# Autodesk Inventor assembly: Box Arm
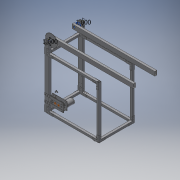
[picture p0: Inventor's stored thumbnail of the model, 180x180]
Saved by Autodesk Inventor 2018 (Build 220112000, 112)
## iProperties
Created: 2019-01-16
Part Number: Box Arm
Document SubType Name: Assembly
Designer: Gabriel
Author: Gabriel
## Documents named in this file (33)
- C:\Users\Gabriel\Documents\GitHub\2019CAD\Drivebase Box Arm\Box Arm.iam
- C:\Users\Gabriel\Documents\GitHub\2019CAD\Drivebase Box Arm\30in 1x1 Beam.ipt
- C:\Users\Gabriel\Documents\GitHub\2019CAD\Drivebase Box Arm\25in 1x1 Beam.ipt
- C:\Users\Gabriel\Documents\GitHub\2019CAD\Drivebase Box Arm\17in 1x1 Beam.ipt
- C:\Users\Gabriel\Documents\GitHub\2019CAD\Drivebase Box Arm\23in 1x1 Beam.ipt
- C:\Users\Gabriel\Documents\GitHub\2019CAD\Drivebase Box Arm\L gusset.ipt
- C:\Users\Gabriel\Documents\GitHub\2019CAD\Drivebase Box Arm\34.48in Arm Bea.ipt
- C:\Users\Gabriel\Documents\GitHub\2019CAD\Drivebase Box Arm\0_500_ID_x_1_125_OD_x_0_313_WD_Flanged_Bearing_217-2731.ipt
- C:\Users\Gabriel\Documents\GitHub\2019CAD\Drivebase Box Arm\_72t_Aluminum_Plate_Sprocket_25_Chain_1-1_8_Bearing_Bore_217-2627.ipt
- C:\Users\Gabriel\Documents\GitHub\2019CAD\Drivebase Box Arm\Hex Hub.ipt
- C:\Users\Gabriel\Documents\GitHub\2019CAD\Drivebase Box Arm\0.5in Hex Shaft.ipt
- C:\Users\Gabriel\Documents\GitHub\2019CAD\Drivebase Box Arm\1_2_Acetal_Spacer_-_1_2_Hex_217-3261.ipt
- C:\Users\Gabriel\Documents\GitHub\2019CAD\Drivebase Box Arm\am-0150 Toughbox Large Output Gear.ipt
- C:\Users\Gabriel\Documents\GitHub\2019CAD\Drivebase Box Arm\Mini_CIM_Motor_217-3371.ipt
- C:\Users\Gabriel\Documents\GitHub\2019CAD\Drivebase Box Arm\ARm Gearbox Plate.ipt
- C:\Users\Gabriel\Documents\GitHub\2019CAD\Drivebase Box Arm\1_16_Acetal_Spacer_-_1_2_Hex_217-3257.ipt
- C:\Users\Gabriel\Documents\GitHub\2019CAD\Drivebase Box Arm\3_8in Hex Shaft.ipt
- C:\Users\Gabriel\Documents\GitHub\2019CAD\Drivebase Box Arm\10T_Steel_Spur_Gear_20_DP_12T_Center_Distance_CIM_Motor_217-6334.ipt
- C:\Users\Gabriel\Documents\GitHub\2019CAD\Drivebase Box Arm\am-0143 50 Tooth 20 dp Aluminum Gear 375 Hex.ipt
- C:\Users\Gabriel\Documents\GitHub\2019CAD\Drivebase Box Arm\am-0151 14T 20dp 375hex.ipt
- C:\Users\Gabriel\Documents\GitHub\2019CAD\Drivebase Box Arm\1_16_Acetal_Spacer_-_3_8_Hex_217-3258.ipt
- C:\Users\Gabriel\Documents\GitHub\2019CAD\Drivebase Box Arm\40t_Aluminum_Spur_Gear_20_DP_3_8_Hex_Bore_217-2707.ipt
- C:\Users\Gabriel\Documents\GitHub\2019CAD\Drivebase Box Arm\am-0028 00.375'' id Flanged, Shielded Ball Bearing (FR6ZZ).ipt
- C:\Users\Gabriel\Documents\GitHub\2019CAD\Drivebase Box Arm\92196A271_18-8 STAINLESS STEEL SOCKET HEAD CAP SCREW.ipt
- C:\Users\Gabriel\Documents\GitHub\2019CAD\Drivebase Box Arm\am-3621 - S25-18HA-500H.ipt
- C:\Users\Gabriel\Documents\GitHub\2019CAD\Drivebase Box Arm\Clamping_Shaft_Collar_-_1_2_Hex_ID_217-2737.ipt
- C:\Users\Gabriel\Documents\GitHub\2019CAD\Drivebase Box Arm\#10 Washer.ipt
- C:\Users\Gabriel\Downloads\3D Model Spacer.ipt
- C:\Users\Gabriel\Downloads\Gearbox Mounting Gusset.ipt
- C:\Users\Gabriel\Downloads\92196A251_18-8 STAINLESS STEEL SOCKET HEAD CAP SCREW.ipt
- C:\Users\Gabriel\Downloads\91831A011_TYPE 18-8 STAINLESS STL NYLON-INSERT LOCKNUT.ipt
- C:\Users\Gabriel\Downloads\Churro For ARm Gearbox.ipt
- C:\Users\Gabriel\Downloads\92196A245_18-8 STAINLESS STEEL SOCKET HEAD CAP SCREW.ipt
## Components (119 placed, 32 different names)
1. 30in 1x1 Beam:1 — Mate:13, Mate:14, Mate:37, Mate:38, Mate:74, Mate:75, Mate:83, Mate:84, Mate:98, Mate:99, Mate:101, Mate:102, Mate:103, Mate:104
2. 30in 1x1 Beam:2 — Mate:11, Mate:12, Mate:39, Mate:40, Mate:73, Mate:76, Mate:86, Mate:87, Mate:95, Mate:96, Mate:105, Mate:106, Mate:107, Mate:108, Mate:441, Mate:442, Mate:457, Mate:458, Mate:459, Mate:460, Mate:461, Mate:462, Mate:497
3. 25in 1x1 Beam:1 — Mate:512, Mate:513, Mate:514, Mate:515, Mate:516, Mate:517, Mate:518, Mate:519, Mate:520, Mate:521
4. 25in 1x1 Beam:2 — Mate:464, Mate:465, Mate:466, Mate:467, Mate:469, Mate:472, Mate:475, Mate:476, Mate:477, Mate:478, Mate:479, Mate:480, Mate:481, Mate:482, Mate:487
5. 25in 1x1 Beam:3 — Mate:496, Mate:497, Mate:498, Mate:499, Mate:500, Mate:501, Mate:502, Mate:503, Mate:504
6. 25in 1x1 Beam:4 — Mate:31, Mate:32, Mate:55, Mate:56, Mate:100, Mate:505, Mate:512
7. 17in 1x1 Beam:1 — Mate:504, Mate:505, Mate:506, Mate:507, Mate:508, Mate:509, Mate:510, Mate:511
8. 17in 1x1 Beam:2 — Mate:21, Mate:22, Mate:23, Mate:24
9. 23in 1x1 Beam:1 — Mate:483, Mate:484, Mate:485, Mate:486, Mate:487, Mate:488, Mate:489, Mate:490, Mate:491, Mate:492, Mate:493, Mate:494, Mate:495
10. 23in 1x1 Beam:2 — Mate:47, Mate:48, Mate:51, Mate:52, Mate:85, Mate:89, Mate:522, Mate:523, Mate:524, Mate:525
11. L gusset:1 — Mate:466, Mate:469, Mate:476, Mate:498, Mate:500, Mate:501, Mate:570, Mate:571
12. L gusset:4 — Mate:465, Mate:477, Mate:478, Mate:479, Mate:483, Mate:488, Mate:489, Mate:526, Mate:527, Mate:566, Mate:567, Mate:568, Mate:569
13. L gusset:5 — Mate:51, Mate:52, Mate:513, Mate:517, Mate:518, Mate:519
14. L gusset:7 — Mate:11, Mate:12, Mate:23, Mate:24
15. L gusset:9 — Mate:13, Mate:14, Mate:21, Mate:22
16. L gusset:11 — Mate:31, Mate:32, Mate:74, Mate:75
17. L gusset:12 — Mate:73, Mate:76, Mate:499, Mate:502, Mate:503
18. L gusset:13 — Mate:485, Mate:490, Mate:491
19. L gusset:14 — Mate:47, Mate:48
20. L gusset:15 — Mate:39, Mate:40, Mate:77, Mate:80
21. L gusset:16 — Mate:37, Mate:38, Mate:78, Mate:79
22. L gusset:17 — Mate:55, Mate:56, Mate:515, Mate:520, Mate:521
23. L gusset:18 — Mate:467, Mate:472, Mate:475, Mate:496, Mate:507, Mate:508, Mate:509
24. L gusset:19 — Mate:506, Mate:510, Mate:511, Mate:516
25. 17in 1x1 Beam:3 — Mate:77, Mate:78, Mate:79, Mate:80
26. 34.48in Arm Bea:2 — Mate:109, Mate:110
27. 0_500_ID_x_1_125_OD_x_0_313_WD_Flanged_Bearing_217-2731:1 — Mate:103, Mate:104, Mate:139, Mate:140, Mate:149
28. 0_500_ID_x_1_125_OD_x_0_313_WD_Flanged_Bearing_217-2731:2 — Mate:107, Mate:108, Mate:126, Mate:152
29. 0_500_ID_x_1_125_OD_x_0_313_WD_Flanged_Bearing_217-2731:5 — Mate:101, Mate:102, Mate:143
30. 0_500_ID_x_1_125_OD_x_0_313_WD_Flanged_Bearing_217-2731:8 — Mate:105, Mate:106, Mate:446, Mate:447
31. L gusset:20 — Mate:464, Mate:480, Mate:481, Mate:482, Mate:484, Mate:494, Mate:495, Mate:557
32. L gusset:21 — Mate:89, Mate:514, Mate:522, Mate:523
33. L gusset:22 — Mate:98, Mate:99, Mate:100
34. L gusset:23 — Mate:95, Mate:96
35. L gusset:24 — Mate:83, Mate:84, Mate:85, Mate:524, Mate:525
36. L gusset:25 — Mate:86, Mate:87, Mate:486, Mate:492, Mate:493
37. _72t_Aluminum_Plate_Sprocket_25_Chain_1-1_8_Bearing_Bore_217-2627:2 — Mate:120, Mate:121, Mate:138, Flush:4
38. Hex Hub:2 — Mate:109, Mate:110, Mate:111, Mate:112, Mate:113
39. Hex Hub:3 — Mate:120, Mate:121, Mate:138, Mate:444, Mate:445
40. 1_2_Acetal_Spacer_-_1_2_Hex_217-3261:1 — Mate:126, Mate:406
41. 1_2_Acetal_Spacer_-_1_2_Hex_217-3261:3 — Mate:111, Mate:112, Mate:113
42. 34.48in Arm Bea:3 — Mate:128
43. Hex Hub:4 — Mate:136, Mate:139, Mate:140
44. Hex Hub:5 — Mate:128, Mate:133
45. 1_2_Acetal_Spacer_-_1_2_Hex_217-3261:7 — Mate:143, Mate:403
46. 1_2_Acetal_Spacer_-_1_2_Hex_217-3261:8 — Mate:133, Mate:136
47. 1_2_Acetal_Spacer_-_1_2_Hex_217-3261:9 — Mate:149
48. 1_2_Acetal_Spacer_-_1_2_Hex_217-3261:10 — Mate:152
49. 0.5in Hex Shaft:5 — Mate:345, Mate:346, Mate:347, Mate:348, Mate:349, Mate:350, Mate:351, Mate:386, Mate:387, Mate:389, Mate:390, Mate:395, Mate:396, Mate:398, Mate:399, Rotation:1, Mate:437, Mate:438, Flush:3, Mate:448, Mate:449
50. Mini_CIM_Motor_217-3371:5 — Mate:431, Mate:432, Mate:433, Mate:434, Mate:435, Mate:436
51. am-0150 Toughbox Large Output Gear:8 — Mate:345, Mate:346, Mate:347, Mate:352
52. 1_16_Acetal_Spacer_-_1_2_Hex_217-3257:4 — Mate:348, Mate:349, Mate:352, Mate:353
53. 1_16_Acetal_Spacer_-_1_2_Hex_217-3257:6 — Mate:350, Mate:351, Mate:353, Mate:354
54. 3_8in Hex Shaft:5 — Mate:313, Mate:314, Mate:315, Mate:316, Mate:317, Mate:318, Mate:321, Mate:322, Mate:357, Mate:358, Mate:411, Flush:2, Mate:425, Rotation:2
55. am-0151 14T 20dp 375hex:1 — Mate:325, Mate:326, Mate:331, Mate:335
56. am-0151 14T 20dp 375hex:3 — Mate:315, Mate:316, Mate:320, Mate:359
57. am-0143 50 Tooth 20 dp Aluminum Gear 375 Hex:5 — Mate:327, Mate:328, Mate:332, Mate:339
58. 10T_Steel_Spur_Gear_20_DP_12T_Center_Distance_CIM_Motor_217-6334:6 — Mate:434, Mate:435, Mate:436
59. 1_16_Acetal_Spacer_-_3_8_Hex_217-3258:2 — Mate:337, Mate:338, Mate:339
60. 1_16_Acetal_Spacer_-_3_8_Hex_217-3258:3 — Mate:333, Mate:334, Mate:335, Mate:422
61. 1_16_Acetal_Spacer_-_3_8_Hex_217-3258:5 — Mate:321, Mate:322, Mate:323, Mate:423
62. 1_16_Acetal_Spacer_-_3_8_Hex_217-3258:6 — Mate:317, Mate:318, Mate:319, Mate:320
63. 40t_Aluminum_Spur_Gear_20_DP_3_8_Hex_Bore_217-2707:1 — Mate:313, Mate:314, Mate:319, Mate:323
64. 3_8in Hex Shaft:10 — Mate:325, Mate:326, Mate:327, Mate:328, Mate:329, Mate:330, Mate:333, Mate:334, Mate:337, Mate:338, Mate:412, Flush:1, Mate:424, Mate:426, Rotation:3
65. ARm Gearbox Plate:5 — Mate:341, Mate:344, Mate:413, Mate:414, Mate:415, Mate:416, Mate:441, Mate:442, Mate:451, Mate:452, Mate:453, Mate:454, Mate:455, Mate:456, Mate:537, Mate:539, Mate:541, Mate:543
66. ARm Gearbox Plate:6 — Mate:342, Mate:343, Mate:360, Mate:361, Mate:362, Mate:363, Mate:407, Mate:408, Mate:409, Mate:410, Mate:419, Mate:421, Rotation:1, Mate:544, Mate:546, Mate:547, Mate:548, Mate:549, Mate:553, Mate:554, Mate:555
67. 1_16_Acetal_Spacer_-_3_8_Hex_217-3258:8 — Mate:357, Mate:358, Mate:359
68. 1_16_Acetal_Spacer_-_3_8_Hex_217-3258:10 — Mate:329, Mate:330, Mate:331, Mate:332
69. 0_500_ID_x_1_125_OD_x_0_313_WD_Flanged_Bearing_217-2731:9 — Mate:341, Mate:344, Mate:439
70. 0_500_ID_x_1_125_OD_x_0_313_WD_Flanged_Bearing_217-2731:10 — Mate:342, Mate:343, Mate:354, Mate:450
71. 92196A271_18-8 STAINLESS STEEL SOCKET HEAD CAP SCREW:1 — Mate:361, Mate:363, Mate:420, Mate:429, Mate:431
72. 92196A271_18-8 STAINLESS STEEL SOCKET HEAD CAP SCREW:2 — Mate:360, Mate:362, Mate:417, Mate:427, Mate:432
73. am-0028 00.375'' id Flanged, Shielded Ball Bearing (FR6ZZ):3 — Mate:414, Mate:416, Mate:425, Rotation:2
74. am-0028 00.375'' id Flanged, Shielded Ball Bearing (FR6ZZ):4 — Mate:413, Mate:415, Mate:424, Mate:426, Rotation:3
75. am-3621 - S25-18HA-500H:1 — Mate:386, Mate:387, Flush:4
76. 1_2_Acetal_Spacer_-_1_2_Hex_217-3261:11 — Mate:389, Mate:390, Mate:397
77. Clamping_Shaft_Collar_-_1_2_Hex_ID_217-2737:1 — Mate:395, Mate:396, Mate:397, Flush:3
78. Clamping_Shaft_Collar_-_1_2_Hex_ID_217-2737:2 — Mate:398, Mate:399, Mate:440
79. Clamping_Shaft_Collar_-_1_2_Hex_ID_217-2737:5 — Mate:406
80. Clamping_Shaft_Collar_-_1_2_Hex_ID_217-2737:6 — Mate:403
81. am-0028 00.375'' id Flanged, Shielded Ball Bearing (FR6ZZ):5 — Mate:409, Mate:410, Mate:411, Flush:2, Mate:423
82. am-0028 00.375'' id Flanged, Shielded Ball Bearing (FR6ZZ):6 — Mate:407, Mate:408, Mate:412, Flush:1, Mate:422
83. #10 Washer:1 — Mate:417, Mate:419, Mate:428
84. #10 Washer:2 — Mate:420, Mate:421, Mate:430
85. #10 Washer:3 — Mate:427, Mate:428, Mate:433
86. #10 Washer:4 — Mate:429, Mate:430
87. 1_16_Acetal_Spacer_-_1_2_Hex_217-3257:9 — Mate:437, Mate:438, Mate:439, Mate:440
88. 1_2_Acetal_Spacer_-_1_2_Hex_217-3261:12 — Mate:444, Mate:445, Mate:446, Mate:447
89. 3D Model Spacer:1 — Mate:448, Mate:449, Mate:450
90. Gearbox Mounting Gusset:1 — Mate:451, Mate:452, Mate:453, Mate:457, Mate:459, Mate:460, Mate:528, Mate:529, Mate:532, Mate:535, Mate:558, Mate:559, Mate:560, Mate:561
91. Gearbox Mounting Gusset:2 — Mate:454, Mate:455, Mate:456, Mate:458, Mate:461, Mate:462, Mate:530, Mate:531, Mate:533, Mate:534, Mate:562, Mate:563, Mate:564, Mate:565
92. 92196A251_18-8 STAINLESS STEEL SOCKET HEAD CAP SCREW:1 — Mate:526, Mate:527, Mate:556
93. 91831A011_TYPE 18-8 STAINLESS STL NYLON-INSERT LOCKNUT:1 — Mate:556, Mate:557
94. 91831A011_TYPE 18-8 STAINLESS STL NYLON-INSERT LOCKNUT:2
95. 91831A011_TYPE 18-8 STAINLESS STL NYLON-INSERT LOCKNUT:3
96. 91831A011_TYPE 18-8 STAINLESS STL NYLON-INSERT LOCKNUT:4
97. Churro For ARm Gearbox:1 — Mate:540, Mate:541, Mate:545
98. Churro For ARm Gearbox:2 — Mate:538, Mate:539, Mate:550
99. Churro For ARm Gearbox:3 — Mate:542, Mate:543, Mate:552
100. Churro For ARm Gearbox:4 — Mate:536, Mate:537, Mate:551
101. 92196A245_18-8 STAINLESS STEEL SOCKET HEAD CAP SCREW:1 — Mate:531, Mate:534, Mate:542
102. 92196A245_18-8 STAINLESS STEEL SOCKET HEAD CAP SCREW:2 — Mate:528, Mate:529, Mate:536
103. 92196A245_18-8 STAINLESS STEEL SOCKET HEAD CAP SCREW:3 — Mate:532, Mate:535, Mate:538
104. 92196A245_18-8 STAINLESS STEEL SOCKET HEAD CAP SCREW:4 — Mate:530, Mate:533, Mate:540
105. 92196A245_18-8 STAINLESS STEEL SOCKET HEAD CAP SCREW:5 — Mate:549, Mate:552, Mate:555
106. 92196A245_18-8 STAINLESS STEEL SOCKET HEAD CAP SCREW:6 — Mate:547, Mate:550, Mate:553
107. 92196A245_18-8 STAINLESS STEEL SOCKET HEAD CAP SCREW:7 — Mate:548, Mate:551, Mate:554
108. 92196A245_18-8 STAINLESS STEEL SOCKET HEAD CAP SCREW:8 — Mate:544, Mate:545, Mate:546
109. 92196A251_18-8 STAINLESS STEEL SOCKET HEAD CAP SCREW:2 — Mate:566
110. 92196A251_18-8 STAINLESS STEEL SOCKET HEAD CAP SCREW:3 — Mate:558, Mate:559
111. 92196A251_18-8 STAINLESS STEEL SOCKET HEAD CAP SCREW:4 — Mate:567
112. 92196A251_18-8 STAINLESS STEEL SOCKET HEAD CAP SCREW:5 — Mate:568
113. 92196A251_18-8 STAINLESS STEEL SOCKET HEAD CAP SCREW:6 — Mate:563, Mate:565
114. 92196A251_18-8 STAINLESS STEEL SOCKET HEAD CAP SCREW:7 — Mate:562, Mate:564
115. 92196A251_18-8 STAINLESS STEEL SOCKET HEAD CAP SCREW:8 — Mate:560, Mate:561
116. 92196A251_18-8 STAINLESS STEEL SOCKET HEAD CAP SCREW:9 — Mate:571
117. 92196A251_18-8 STAINLESS STEEL SOCKET HEAD CAP SCREW:10 — Mate:570
118. 92196A251_18-8 STAINLESS STEEL SOCKET HEAD CAP SCREW:11
119. 92196A251_18-8 STAINLESS STEEL SOCKET HEAD CAP SCREW:12 — Mate:569
## Relationships (285: Mate 278, Flush 4, RelateRotation 3)
- Mate:11: 30in 1x1 Beam:2 ↔ L gusset:7
- Mate:12: 30in 1x1 Beam:2 ↔ L gusset:7
- Mate:13: 30in 1x1 Beam:1 ↔ L gusset:9
- Mate:14: 30in 1x1 Beam:1 ↔ L gusset:9
- Mate:21: 17in 1x1 Beam:2 ↔ L gusset:9
- Mate:22: 17in 1x1 Beam:2 ↔ L gusset:9
- Mate:23: 17in 1x1 Beam:2 ↔ L gusset:7
- Mate:24: 17in 1x1 Beam:2 ↔ L gusset:7
- Mate:31: 25in 1x1 Beam:4 ↔ L gusset:11
- Mate:32: 25in 1x1 Beam:4 ↔ L gusset:11
- Mate:37: 30in 1x1 Beam:1 ↔ L gusset:16
- Mate:38: 30in 1x1 Beam:1 ↔ L gusset:16
- Mate:39: 30in 1x1 Beam:2 ↔ L gusset:15
- Mate:40: 30in 1x1 Beam:2 ↔ L gusset:15
- Mate:47: 23in 1x1 Beam:2 ↔ L gusset:14
- Mate:48: 23in 1x1 Beam:2 ↔ L gusset:14
- Mate:51: 23in 1x1 Beam:2 ↔ L gusset:5
- Mate:52: 23in 1x1 Beam:2 ↔ L gusset:5
- Mate:55: 25in 1x1 Beam:4 ↔ L gusset:17
- Mate:56: 25in 1x1 Beam:4 ↔ L gusset:17
- Mate:73: 30in 1x1 Beam:2 ↔ L gusset:12
- Mate:74: 30in 1x1 Beam:1 ↔ L gusset:11
- Mate:75: 30in 1x1 Beam:1 ↔ L gusset:11
- Mate:76: 30in 1x1 Beam:2 ↔ L gusset:12
- Mate:77: L gusset:15 ↔ 17in 1x1 Beam:3
- Mate:78: L gusset:16 ↔ 17in 1x1 Beam:3
- Mate:79: L gusset:16 ↔ 17in 1x1 Beam:3
- Mate:80: L gusset:15 ↔ 17in 1x1 Beam:3
- Mate:83: 30in 1x1 Beam:1 ↔ L gusset:24
- Mate:84: 30in 1x1 Beam:1 ↔ L gusset:24
- Mate:85: 23in 1x1 Beam:2 ↔ L gusset:24
- Mate:86: 30in 1x1 Beam:2 ↔ L gusset:25
- Mate:87: 30in 1x1 Beam:2 ↔ L gusset:25
- Mate:89: 23in 1x1 Beam:2 ↔ L gusset:21
- Mate:95: 30in 1x1 Beam:2 ↔ L gusset:23
- Mate:96: 30in 1x1 Beam:2 ↔ L gusset:23
- Mate:98: 30in 1x1 Beam:1 ↔ L gusset:22
- Mate:99: 30in 1x1 Beam:1 ↔ L gusset:22
- Mate:100: 25in 1x1 Beam:4 ↔ L gusset:22
- Mate:101: 30in 1x1 Beam:1 ↔ 0_500_ID_x_1_125_OD_x_0_313_WD_Flanged_Bearing_217-2731:5
- Mate:102: 30in 1x1 Beam:1 ↔ 0_500_ID_x_1_125_OD_x_0_313_WD_Flanged_Bearing_217-2731:5
- Mate:103: 30in 1x1 Beam:1 ↔ 0_500_ID_x_1_125_OD_x_0_313_WD_Flanged_Bearing_217-2731:1
- Mate:104: 30in 1x1 Beam:1 ↔ 0_500_ID_x_1_125_OD_x_0_313_WD_Flanged_Bearing_217-2731:1
- Mate:105: 30in 1x1 Beam:2 ↔ 0_500_ID_x_1_125_OD_x_0_313_WD_Flanged_Bearing_217-2731:8
- Mate:106: 30in 1x1 Beam:2 ↔ 0_500_ID_x_1_125_OD_x_0_313_WD_Flanged_Bearing_217-2731:8
- Mate:107: 30in 1x1 Beam:2 ↔ 0_500_ID_x_1_125_OD_x_0_313_WD_Flanged_Bearing_217-2731:2
- Mate:108: 30in 1x1 Beam:2 ↔ 0_500_ID_x_1_125_OD_x_0_313_WD_Flanged_Bearing_217-2731:2
- Mate:109: 34.48in Arm Bea:2 ↔ Hex Hub:2
- Mate:110: 34.48in Arm Bea:2 ↔ Hex Hub:2
- Mate:111: Hex Hub:2 ↔ 1_2_Acetal_Spacer_-_1_2_Hex_217-3261:3
- Mate:112: Hex Hub:2 ↔ 1_2_Acetal_Spacer_-_1_2_Hex_217-3261:3
- Mate:113: Hex Hub:2 ↔ 1_2_Acetal_Spacer_-_1_2_Hex_217-3261:3
- Mate:120: _72t_Aluminum_Plate_Sprocket_25_Chain_1-1_8_Bearing_Bore_217-2627:2 ↔ Hex Hub:3
- Mate:121: _72t_Aluminum_Plate_Sprocket_25_Chain_1-1_8_Bearing_Bore_217-2627:2 ↔ Hex Hub:3
- Mate:126: 0_500_ID_x_1_125_OD_x_0_313_WD_Flanged_Bearing_217-2731:2 ↔ 1_2_Acetal_Spacer_-_1_2_Hex_217-3261:1
- Mate:128: 34.48in Arm Bea:3 ↔ Hex Hub:5
- Mate:133: Hex Hub:5 ↔ 1_2_Acetal_Spacer_-_1_2_Hex_217-3261:8
- Mate:136: Hex Hub:4 ↔ 1_2_Acetal_Spacer_-_1_2_Hex_217-3261:8
- Mate:138: _72t_Aluminum_Plate_Sprocket_25_Chain_1-1_8_Bearing_Bore_217-2627:2 ↔ Hex Hub:3
- Mate:139: 0_500_ID_x_1_125_OD_x_0_313_WD_Flanged_Bearing_217-2731:1 ↔ Hex Hub:4
- Mate:140: 0_500_ID_x_1_125_OD_x_0_313_WD_Flanged_Bearing_217-2731:1 ↔ Hex Hub:4
- Mate:143: 0_500_ID_x_1_125_OD_x_0_313_WD_Flanged_Bearing_217-2731:5 ↔ 1_2_Acetal_Spacer_-_1_2_Hex_217-3261:7
- Mate:149: 0_500_ID_x_1_125_OD_x_0_313_WD_Flanged_Bearing_217-2731:1 ↔ 1_2_Acetal_Spacer_-_1_2_Hex_217-3261:9
- Mate:152: 0_500_ID_x_1_125_OD_x_0_313_WD_Flanged_Bearing_217-2731:2 ↔ 1_2_Acetal_Spacer_-_1_2_Hex_217-3261:10
- Mate:313: 3_8in Hex Shaft:5 ↔ 40t_Aluminum_Spur_Gear_20_DP_3_8_Hex_Bore_217-2707:1
- Mate:314: 3_8in Hex Shaft:5 ↔ 40t_Aluminum_Spur_Gear_20_DP_3_8_Hex_Bore_217-2707:1
- Mate:315: 3_8in Hex Shaft:5 ↔ am-0151 14T 20dp 375hex:3
- Mate:316: 3_8in Hex Shaft:5 ↔ am-0151 14T 20dp 375hex:3
- Mate:317: 3_8in Hex Shaft:5 ↔ 1_16_Acetal_Spacer_-_3_8_Hex_217-3258:6
- Mate:318: 3_8in Hex Shaft:5 ↔ 1_16_Acetal_Spacer_-_3_8_Hex_217-3258:6
- Mate:319: 1_16_Acetal_Spacer_-_3_8_Hex_217-3258:6 ↔ 40t_Aluminum_Spur_Gear_20_DP_3_8_Hex_Bore_217-2707:1
- Mate:320: am-0151 14T 20dp 375hex:3 ↔ 1_16_Acetal_Spacer_-_3_8_Hex_217-3258:6
- Mate:321: 3_8in Hex Shaft:5 ↔ 1_16_Acetal_Spacer_-_3_8_Hex_217-3258:5
- Mate:322: 3_8in Hex Shaft:5 ↔ 1_16_Acetal_Spacer_-_3_8_Hex_217-3258:5
- Mate:323: 1_16_Acetal_Spacer_-_3_8_Hex_217-3258:5 ↔ 40t_Aluminum_Spur_Gear_20_DP_3_8_Hex_Bore_217-2707:1
- Mate:325: am-0151 14T 20dp 375hex:1 ↔ 3_8in Hex Shaft:10
- Mate:326: am-0151 14T 20dp 375hex:1 ↔ 3_8in Hex Shaft:10
- Mate:327: am-0143 50 Tooth 20 dp Aluminum Gear 375 Hex:5 ↔ 3_8in Hex Shaft:10
- Mate:328: am-0143 50 Tooth 20 dp Aluminum Gear 375 Hex:5 ↔ 3_8in Hex Shaft:10
- Mate:329: 3_8in Hex Shaft:10 ↔ 1_16_Acetal_Spacer_-_3_8_Hex_217-3258:10
- Mate:330: 3_8in Hex Shaft:10 ↔ 1_16_Acetal_Spacer_-_3_8_Hex_217-3258:10
- Mate:331: am-0151 14T 20dp 375hex:1 ↔ 1_16_Acetal_Spacer_-_3_8_Hex_217-3258:10
- Mate:332: am-0143 50 Tooth 20 dp Aluminum Gear 375 Hex:5 ↔ 1_16_Acetal_Spacer_-_3_8_Hex_217-3258:10
- Mate:333: 1_16_Acetal_Spacer_-_3_8_Hex_217-3258:3 ↔ 3_8in Hex Shaft:10
- Mate:334: 1_16_Acetal_Spacer_-_3_8_Hex_217-3258:3 ↔ 3_8in Hex Shaft:10
- Mate:335: am-0151 14T 20dp 375hex:1 ↔ 1_16_Acetal_Spacer_-_3_8_Hex_217-3258:3
- Mate:337: 1_16_Acetal_Spacer_-_3_8_Hex_217-3258:2 ↔ 3_8in Hex Shaft:10
- Mate:338: 1_16_Acetal_Spacer_-_3_8_Hex_217-3258:2 ↔ 3_8in Hex Shaft:10
- Mate:339: am-0143 50 Tooth 20 dp Aluminum Gear 375 Hex:5 ↔ 1_16_Acetal_Spacer_-_3_8_Hex_217-3258:2
- Mate:341: ARm Gearbox Plate:5 ↔ 0_500_ID_x_1_125_OD_x_0_313_WD_Flanged_Bearing_217-2731:9
- Mate:342: ARm Gearbox Plate:6 ↔ 0_500_ID_x_1_125_OD_x_0_313_WD_Flanged_Bearing_217-2731:10
- Mate:343: ARm Gearbox Plate:6 ↔ 0_500_ID_x_1_125_OD_x_0_313_WD_Flanged_Bearing_217-2731:10
- Mate:344: ARm Gearbox Plate:5 ↔ 0_500_ID_x_1_125_OD_x_0_313_WD_Flanged_Bearing_217-2731:9
- Mate:345: 0.5in Hex Shaft:5 ↔ am-0150 Toughbox Large Output Gear:8
- Mate:346: 0.5in Hex Shaft:5 ↔ am-0150 Toughbox Large Output Gear:8
- Mate:347: 0.5in Hex Shaft:5 ↔ am-0150 Toughbox Large Output Gear:8
- Mate:348: 0.5in Hex Shaft:5 ↔ 1_16_Acetal_Spacer_-_1_2_Hex_217-3257:4
- Mate:349: 0.5in Hex Shaft:5 ↔ 1_16_Acetal_Spacer_-_1_2_Hex_217-3257:4
- Mate:350: 0.5in Hex Shaft:5 ↔ 1_16_Acetal_Spacer_-_1_2_Hex_217-3257:6
- Mate:351: 0.5in Hex Shaft:5 ↔ 1_16_Acetal_Spacer_-_1_2_Hex_217-3257:6
- Mate:352: am-0150 Toughbox Large Output Gear:8 ↔ 1_16_Acetal_Spacer_-_1_2_Hex_217-3257:4
- Mate:353: 1_16_Acetal_Spacer_-_1_2_Hex_217-3257:4 ↔ 1_16_Acetal_Spacer_-_1_2_Hex_217-3257:6
- Mate:354: 1_16_Acetal_Spacer_-_1_2_Hex_217-3257:6 ↔ 0_500_ID_x_1_125_OD_x_0_313_WD_Flanged_Bearing_217-2731:10
- Mate:357: 3_8in Hex Shaft:5 ↔ 1_16_Acetal_Spacer_-_3_8_Hex_217-3258:8
- Mate:358: 3_8in Hex Shaft:5 ↔ 1_16_Acetal_Spacer_-_3_8_Hex_217-3258:8
- Mate:359: am-0151 14T 20dp 375hex:3 ↔ 1_16_Acetal_Spacer_-_3_8_Hex_217-3258:8
- Mate:360: ARm Gearbox Plate:6 ↔ 92196A271_18-8 STAINLESS STEEL SOCKET HEAD CAP SCREW:2
- Mate:361: ARm Gearbox Plate:6 ↔ 92196A271_18-8 STAINLESS STEEL SOCKET HEAD CAP SCREW:1
- Mate:362: ARm Gearbox Plate:6 ↔ 92196A271_18-8 STAINLESS STEEL SOCKET HEAD CAP SCREW:2
- Mate:363: ARm Gearbox Plate:6 ↔ 92196A271_18-8 STAINLESS STEEL SOCKET HEAD CAP SCREW:1
- Mate:386: 0.5in Hex Shaft:5 ↔ am-3621 - S25-18HA-500H:1
- Mate:387: 0.5in Hex Shaft:5 ↔ am-3621 - S25-18HA-500H:1
- Mate:389: 0.5in Hex Shaft:5 ↔ 1_2_Acetal_Spacer_-_1_2_Hex_217-3261:11
- Mate:390: 0.5in Hex Shaft:5 ↔ 1_2_Acetal_Spacer_-_1_2_Hex_217-3261:11
- Mate:395: 0.5in Hex Shaft:5 ↔ Clamping_Shaft_Collar_-_1_2_Hex_ID_217-2737:1
- Mate:396: 0.5in Hex Shaft:5 ↔ Clamping_Shaft_Collar_-_1_2_Hex_ID_217-2737:1
- Mate:397: 1_2_Acetal_Spacer_-_1_2_Hex_217-3261:11 ↔ Clamping_Shaft_Collar_-_1_2_Hex_ID_217-2737:1
- Mate:398: 0.5in Hex Shaft:5 ↔ Clamping_Shaft_Collar_-_1_2_Hex_ID_217-2737:2
- Mate:399: 0.5in Hex Shaft:5 ↔ Clamping_Shaft_Collar_-_1_2_Hex_ID_217-2737:2
- Mate:403: 1_2_Acetal_Spacer_-_1_2_Hex_217-3261:7 ↔ Clamping_Shaft_Collar_-_1_2_Hex_ID_217-2737:6
- Mate:406: 1_2_Acetal_Spacer_-_1_2_Hex_217-3261:1 ↔ Clamping_Shaft_Collar_-_1_2_Hex_ID_217-2737:5
- Mate:407: ARm Gearbox Plate:6 ↔ am-0028 00.375'' id Flanged, Shielded Ball Bearing (FR6ZZ):6
- Mate:408: ARm Gearbox Plate:6 ↔ am-0028 00.375'' id Flanged, Shielded Ball Bearing (FR6ZZ):6
- Mate:409: ARm Gearbox Plate:6 ↔ am-0028 00.375'' id Flanged, Shielded Ball Bearing (FR6ZZ):5
- Mate:410: ARm Gearbox Plate:6 ↔ am-0028 00.375'' id Flanged, Shielded Ball Bearing (FR6ZZ):5
- Mate:411: 3_8in Hex Shaft:5 ↔ am-0028 00.375'' id Flanged, Shielded Ball Bearing (FR6ZZ):5
- Mate:412: 3_8in Hex Shaft:10 ↔ am-0028 00.375'' id Flanged, Shielded Ball Bearing (FR6ZZ):6
- Mate:413: ARm Gearbox Plate:5 ↔ am-0028 00.375'' id Flanged, Shielded Ball Bearing (FR6ZZ):4
- Mate:414: ARm Gearbox Plate:5 ↔ am-0028 00.375'' id Flanged, Shielded Ball Bearing (FR6ZZ):3
- Mate:415: ARm Gearbox Plate:5 ↔ am-0028 00.375'' id Flanged, Shielded Ball Bearing (FR6ZZ):4
- Mate:416: ARm Gearbox Plate:5 ↔ am-0028 00.375'' id Flanged, Shielded Ball Bearing (FR6ZZ):3
- Mate:417: 92196A271_18-8 STAINLESS STEEL SOCKET HEAD CAP SCREW:2 ↔ #10 Washer:1
- Mate:419: ARm Gearbox Plate:6 ↔ #10 Washer:1
- Mate:420: 92196A271_18-8 STAINLESS STEEL SOCKET HEAD CAP SCREW:1 ↔ #10 Washer:2
- Mate:421: ARm Gearbox Plate:6 ↔ #10 Washer:2
- Flush:1: 3_8in Hex Shaft:10 ↔ am-0028 00.375'' id Flanged, Shielded Ball Bearing (FR6ZZ):6
- Flush:2: 3_8in Hex Shaft:5 ↔ am-0028 00.375'' id Flanged, Shielded Ball Bearing (FR6ZZ):5
- Rotation:1 [RelateRotation] (1 ul): 0.5in Hex Shaft:5 ↔ ARm Gearbox Plate:6
- Mate:422: 1_16_Acetal_Spacer_-_3_8_Hex_217-3258:3 ↔ am-0028 00.375'' id Flanged, Shielded Ball Bearing (FR6ZZ):6
- Mate:423: 1_16_Acetal_Spacer_-_3_8_Hex_217-3258:5 ↔ am-0028 00.375'' id Flanged, Shielded Ball Bearing (FR6ZZ):5
- Mate:424: 3_8in Hex Shaft:10 ↔ am-0028 00.375'' id Flanged, Shielded Ball Bearing (FR6ZZ):4
- Mate:425: 3_8in Hex Shaft:5 ↔ am-0028 00.375'' id Flanged, Shielded Ball Bearing (FR6ZZ):3
- Mate:426: 3_8in Hex Shaft:10 ↔ am-0028 00.375'' id Flanged, Shielded Ball Bearing (FR6ZZ):4
- Rotation:2 [RelateRotation] (1 ul): 3_8in Hex Shaft:5 ↔ am-0028 00.375'' id Flanged, Shielded Ball Bearing (FR6ZZ):3
- Rotation:3 [RelateRotation] (1 ul): 3_8in Hex Shaft:10 ↔ am-0028 00.375'' id Flanged, Shielded Ball Bearing (FR6ZZ):4
- Mate:427: 92196A271_18-8 STAINLESS STEEL SOCKET HEAD CAP SCREW:2 ↔ #10 Washer:3
- Mate:428: #10 Washer:1 ↔ #10 Washer:3
- Mate:429: 92196A271_18-8 STAINLESS STEEL SOCKET HEAD CAP SCREW:1 ↔ #10 Washer:4
- Mate:430: #10 Washer:2 ↔ #10 Washer:4
- Mate:431: Mini_CIM_Motor_217-3371:5 ↔ 92196A271_18-8 STAINLESS STEEL SOCKET HEAD CAP SCREW:1
- Mate:432: Mini_CIM_Motor_217-3371:5 ↔ 92196A271_18-8 STAINLESS STEEL SOCKET HEAD CAP SCREW:2
- Mate:433: Mini_CIM_Motor_217-3371:5 ↔ #10 Washer:3
- Mate:434: Mini_CIM_Motor_217-3371:5 ↔ 10T_Steel_Spur_Gear_20_DP_12T_Center_Distance_CIM_Motor_217-6334:6
- Mate:435: Mini_CIM_Motor_217-3371:5 ↔ 10T_Steel_Spur_Gear_20_DP_12T_Center_Distance_CIM_Motor_217-6334:6
- Mate:436: Mini_CIM_Motor_217-3371:5 ↔ 10T_Steel_Spur_Gear_20_DP_12T_Center_Distance_CIM_Motor_217-6334:6
- Mate:437: 0.5in Hex Shaft:5 ↔ 1_16_Acetal_Spacer_-_1_2_Hex_217-3257:9
- Mate:438: 0.5in Hex Shaft:5 ↔ 1_16_Acetal_Spacer_-_1_2_Hex_217-3257:9
- Mate:439: 0_500_ID_x_1_125_OD_x_0_313_WD_Flanged_Bearing_217-2731:9 ↔ 1_16_Acetal_Spacer_-_1_2_Hex_217-3257:9
- Mate:440: Clamping_Shaft_Collar_-_1_2_Hex_ID_217-2737:2 ↔ 1_16_Acetal_Spacer_-_1_2_Hex_217-3257:9
- Flush:3: 0.5in Hex Shaft:5 ↔ Clamping_Shaft_Collar_-_1_2_Hex_ID_217-2737:1
- Mate:441: 30in 1x1 Beam:2 ↔ ARm Gearbox Plate:5
- Mate:442: 30in 1x1 Beam:2 ↔ ARm Gearbox Plate:5
- Flush:4: _72t_Aluminum_Plate_Sprocket_25_Chain_1-1_8_Bearing_Bore_217-2627:2 ↔ am-3621 - S25-18HA-500H:1
- Mate:444: Hex Hub:3 ↔ 1_2_Acetal_Spacer_-_1_2_Hex_217-3261:12
- Mate:445: Hex Hub:3 ↔ 1_2_Acetal_Spacer_-_1_2_Hex_217-3261:12
- Mate:446: 0_500_ID_x_1_125_OD_x_0_313_WD_Flanged_Bearing_217-2731:8 ↔ 1_2_Acetal_Spacer_-_1_2_Hex_217-3261:12
- Mate:447: 0_500_ID_x_1_125_OD_x_0_313_WD_Flanged_Bearing_217-2731:8 ↔ 1_2_Acetal_Spacer_-_1_2_Hex_217-3261:12
- Mate:448: 0.5in Hex Shaft:5 ↔ 3D Model Spacer:1
- Mate:449: 0.5in Hex Shaft:5 ↔ 3D Model Spacer:1
- Mate:450: 0_500_ID_x_1_125_OD_x_0_313_WD_Flanged_Bearing_217-2731:10 ↔ 3D Model Spacer:1
- Mate:451: ARm Gearbox Plate:5 ↔ Gearbox Mounting Gusset:1
- Mate:452: ARm Gearbox Plate:5 ↔ Gearbox Mounting Gusset:1
- Mate:453: ARm Gearbox Plate:5 ↔ Gearbox Mounting Gusset:1
- Mate:454: ARm Gearbox Plate:5 ↔ Gearbox Mounting Gusset:2
- Mate:455: ARm Gearbox Plate:5 ↔ Gearbox Mounting Gusset:2
- Mate:456: ARm Gearbox Plate:5 ↔ Gearbox Mounting Gusset:2
- Mate:457: 30in 1x1 Beam:2 ↔ Gearbox Mounting Gusset:1
- Mate:458: 30in 1x1 Beam:2 ↔ Gearbox Mounting Gusset:2
- Mate:459: 30in 1x1 Beam:2 ↔ Gearbox Mounting Gusset:1
- Mate:460: 30in 1x1 Beam:2 ↔ Gearbox Mounting Gusset:1
- Mate:461: 30in 1x1 Beam:2 ↔ Gearbox Mounting Gusset:2
- Mate:462: 30in 1x1 Beam:2 ↔ Gearbox Mounting Gusset:2
- Mate:464: 25in 1x1 Beam:2 ↔ L gusset:20
- Mate:465: 25in 1x1 Beam:2 ↔ L gusset:4
- Mate:466: 25in 1x1 Beam:2 ↔ L gusset:1
- Mate:467: 25in 1x1 Beam:2 ↔ L gusset:18
- Mate:469: 25in 1x1 Beam:2 ↔ L gusset:1
- Mate:472: 25in 1x1 Beam:2 ↔ L gusset:18
- Mate:475: 25in 1x1 Beam:2 ↔ L gusset:18
- Mate:476: 25in 1x1 Beam:2 ↔ L gusset:1
- Mate:477: 25in 1x1 Beam:2 ↔ L gusset:4
- Mate:478: 25in 1x1 Beam:2 ↔ L gusset:4
- Mate:479: 25in 1x1 Beam:2 ↔ L gusset:4
- Mate:480: 25in 1x1 Beam:2 ↔ L gusset:20
- Mate:481: 25in 1x1 Beam:2 ↔ L gusset:20
- Mate:482: 25in 1x1 Beam:2 ↔ L gusset:20
- Mate:483: 23in 1x1 Beam:1 ↔ L gusset:4
- Mate:484: 23in 1x1 Beam:1 ↔ L gusset:20
- Mate:485: 23in 1x1 Beam:1 ↔ L gusset:13
- Mate:486: 23in 1x1 Beam:1 ↔ L gusset:25
- Mate:487: 25in 1x1 Beam:2 ↔ 23in 1x1 Beam:1
- Mate:488: 23in 1x1 Beam:1 ↔ L gusset:4
- Mate:489: 23in 1x1 Beam:1 ↔ L gusset:4
- Mate:490: 23in 1x1 Beam:1 ↔ L gusset:13
- Mate:491: 23in 1x1 Beam:1 ↔ L gusset:13
- Mate:492: 23in 1x1 Beam:1 ↔ L gusset:25
- Mate:493: 23in 1x1 Beam:1 ↔ L gusset:25
- Mate:494: 23in 1x1 Beam:1 ↔ L gusset:20
- Mate:495: 23in 1x1 Beam:1 ↔ L gusset:20
- Mate:496: 25in 1x1 Beam:3 ↔ L gusset:18
- Mate:497: 30in 1x1 Beam:2 ↔ 25in 1x1 Beam:3
- Mate:498: 25in 1x1 Beam:3 ↔ L gusset:1
- Mate:499: 25in 1x1 Beam:3 ↔ L gusset:12
- Mate:500: 25in 1x1 Beam:3 ↔ L gusset:1
- Mate:501: 25in 1x1 Beam:3 ↔ L gusset:1
- Mate:502: 25in 1x1 Beam:3 ↔ L gusset:12
- Mate:503: 25in 1x1 Beam:3 ↔ L gusset:12
- Mate:504: 25in 1x1 Beam:3 ↔ 17in 1x1 Beam:1
- Mate:505: 25in 1x1 Beam:4 ↔ 17in 1x1 Beam:1
- Mate:506: 17in 1x1 Beam:1 ↔ L gusset:19
- Mate:507: 17in 1x1 Beam:1 ↔ L gusset:18
- Mate:508: 17in 1x1 Beam:1 ↔ L gusset:18
- Mate:509: 17in 1x1 Beam:1 ↔ L gusset:18
- Mate:510: 17in 1x1 Beam:1 ↔ L gusset:19
- Mate:511: 17in 1x1 Beam:1 ↔ L gusset:19
- Mate:512: 25in 1x1 Beam:1 ↔ 25in 1x1 Beam:4
- Mate:513: 25in 1x1 Beam:1 ↔ L gusset:5
- Mate:514: 25in 1x1 Beam:1 ↔ L gusset:21
- Mate:515: 25in 1x1 Beam:1 ↔ L gusset:17
- Mate:516: 25in 1x1 Beam:1 ↔ L gusset:19
- Mate:517: 25in 1x1 Beam:1 ↔ L gusset:5
- Mate:518: 25in 1x1 Beam:1 ↔ L gusset:5
- Mate:519: 25in 1x1 Beam:1 ↔ L gusset:5
- Mate:520: 25in 1x1 Beam:1 ↔ L gusset:17
- Mate:521: 25in 1x1 Beam:1 ↔ L gusset:17
- Mate:522: 23in 1x1 Beam:2 ↔ L gusset:21
- Mate:523: 23in 1x1 Beam:2 ↔ L gusset:21
- Mate:524: 23in 1x1 Beam:2 ↔ L gusset:24
- Mate:525: 23in 1x1 Beam:2 ↔ L gusset:24
- Mate:526: L gusset:4 ↔ 92196A251_18-8 STAINLESS STEEL SOCKET HEAD CAP SCREW:1
- Mate:527: L gusset:4 ↔ 92196A251_18-8 STAINLESS STEEL SOCKET HEAD CAP SCREW:1
- Mate:528: Gearbox Mounting Gusset:1 ↔ 92196A245_18-8 STAINLESS STEEL SOCKET HEAD CAP SCREW:2
- Mate:529: Gearbox Mounting Gusset:1 ↔ 92196A245_18-8 STAINLESS STEEL SOCKET HEAD CAP SCREW:2
- Mate:530: Gearbox Mounting Gusset:2 ↔ 92196A245_18-8 STAINLESS STEEL SOCKET HEAD CAP SCREW:4
- Mate:531: Gearbox Mounting Gusset:2 ↔ 92196A245_18-8 STAINLESS STEEL SOCKET HEAD CAP SCREW:1
- Mate:532: Gearbox Mounting Gusset:1 ↔ 92196A245_18-8 STAINLESS STEEL SOCKET HEAD CAP SCREW:3
- Mate:533: Gearbox Mounting Gusset:2 ↔ 92196A245_18-8 STAINLESS STEEL SOCKET HEAD CAP SCREW:4
- Mate:534: Gearbox Mounting Gusset:2 ↔ 92196A245_18-8 STAINLESS STEEL SOCKET HEAD CAP SCREW:1
- Mate:535: Gearbox Mounting Gusset:1 ↔ 92196A245_18-8 STAINLESS STEEL SOCKET HEAD CAP SCREW:3
- Mate:536: Churro For ARm Gearbox:4 ↔ 92196A245_18-8 STAINLESS STEEL SOCKET HEAD CAP SCREW:2
- Mate:537: ARm Gearbox Plate:5 ↔ Churro For ARm Gearbox:4
- Mate:538: Churro For ARm Gearbox:2 ↔ 92196A245_18-8 STAINLESS STEEL SOCKET HEAD CAP SCREW:3
- Mate:539: ARm Gearbox Plate:5 ↔ Churro For ARm Gearbox:2
- Mate:540: Churro For ARm Gearbox:1 ↔ 92196A245_18-8 STAINLESS STEEL SOCKET HEAD CAP SCREW:4
- Mate:541: ARm Gearbox Plate:5 ↔ Churro For ARm Gearbox:1
- Mate:542: Churro For ARm Gearbox:3 ↔ 92196A245_18-8 STAINLESS STEEL SOCKET HEAD CAP SCREW:1
- Mate:543: ARm Gearbox Plate:5 ↔ Churro For ARm Gearbox:3
- Mate:544: ARm Gearbox Plate:6 ↔ 92196A245_18-8 STAINLESS STEEL SOCKET HEAD CAP SCREW:8
- Mate:545: Churro For ARm Gearbox:1 ↔ 92196A245_18-8 STAINLESS STEEL SOCKET HEAD CAP SCREW:8
- Mate:546: ARm Gearbox Plate:6 ↔ 92196A245_18-8 STAINLESS STEEL SOCKET HEAD CAP SCREW:8
- Mate:547: ARm Gearbox Plate:6 ↔ 92196A245_18-8 STAINLESS STEEL SOCKET HEAD CAP SCREW:6
- Mate:548: ARm Gearbox Plate:6 ↔ 92196A245_18-8 STAINLESS STEEL SOCKET HEAD CAP SCREW:7
- Mate:549: ARm Gearbox Plate:6 ↔ 92196A245_18-8 STAINLESS STEEL SOCKET HEAD CAP SCREW:5
- Mate:550: Churro For ARm Gearbox:2 ↔ 92196A245_18-8 STAINLESS STEEL SOCKET HEAD CAP SCREW:6
- Mate:551: Churro For ARm Gearbox:4 ↔ 92196A245_18-8 STAINLESS STEEL SOCKET HEAD CAP SCREW:7
- Mate:552: Churro For ARm Gearbox:3 ↔ 92196A245_18-8 STAINLESS STEEL SOCKET HEAD CAP SCREW:5
- Mate:553: ARm Gearbox Plate:6 ↔ 92196A245_18-8 STAINLESS STEEL SOCKET HEAD CAP SCREW:6
- Mate:554: ARm Gearbox Plate:6 ↔ 92196A245_18-8 STAINLESS STEEL SOCKET HEAD CAP SCREW:7
- Mate:555: ARm Gearbox Plate:6 ↔ 92196A245_18-8 STAINLESS STEEL SOCKET HEAD CAP SCREW:5
- Mate:556: 92196A251_18-8 STAINLESS STEEL SOCKET HEAD CAP SCREW:1 ↔ 91831A011_TYPE 18-8 STAINLESS STL NYLON-INSERT LOCKNUT:1
- Mate:557: L gusset:20 ↔ 91831A011_TYPE 18-8 STAINLESS STL NYLON-INSERT LOCKNUT:1
- Mate:558: Gearbox Mounting Gusset:1 ↔ 92196A251_18-8 STAINLESS STEEL SOCKET HEAD CAP SCREW:3
- Mate:559: Gearbox Mounting Gusset:1 ↔ 92196A251_18-8 STAINLESS STEEL SOCKET HEAD CAP SCREW:3
- Mate:560: Gearbox Mounting Gusset:1 ↔ 92196A251_18-8 STAINLESS STEEL SOCKET HEAD CAP SCREW:8
- Mate:561: Gearbox Mounting Gusset:1 ↔ 92196A251_18-8 STAINLESS STEEL SOCKET HEAD CAP SCREW:8
- Mate:562: Gearbox Mounting Gusset:2 ↔ 92196A251_18-8 STAINLESS STEEL SOCKET HEAD CAP SCREW:7
- Mate:563: Gearbox Mounting Gusset:2 ↔ 92196A251_18-8 STAINLESS STEEL SOCKET HEAD CAP SCREW:6
- Mate:564: Gearbox Mounting Gusset:2 ↔ 92196A251_18-8 STAINLESS STEEL SOCKET HEAD CAP SCREW:7
- Mate:565: Gearbox Mounting Gusset:2 ↔ 92196A251_18-8 STAINLESS STEEL SOCKET HEAD CAP SCREW:6
- Mate:566: L gusset:4 ↔ 92196A251_18-8 STAINLESS STEEL SOCKET HEAD CAP SCREW:2
- Mate:567: L gusset:4 ↔ 92196A251_18-8 STAINLESS STEEL SOCKET HEAD CAP SCREW:4
- Mate:568: L gusset:4 ↔ 92196A251_18-8 STAINLESS STEEL SOCKET HEAD CAP SCREW:5
- Mate:569: L gusset:4 ↔ 92196A251_18-8 STAINLESS STEEL SOCKET HEAD CAP SCREW:12
- Mate:570: L gusset:1 ↔ 92196A251_18-8 STAINLESS STEEL SOCKET HEAD CAP SCREW:10
- Mate:571: L gusset:1 ↔ 92196A251_18-8 STAINLESS STEEL SOCKET HEAD CAP SCREW:9
